# Autodesk Inventor assembly: b5
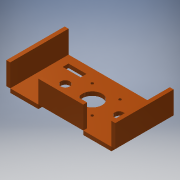
[picture p0: Inventor's stored thumbnail of the model, 180x180]
Saved by Autodesk Inventor 2017 (Build 210142000, 142)
## iProperties
Created: 2016-06-11
Part Number: b5
Document SubType Name: Assembly
Designer: daniel
Author: daniel
## Documents named in this file (4)
- C:\Users\daniel\Documents\GitHub\cardboard-stage-metric\stage\b5.iam
- C:\Users\daniel\Documents\GitHub\cardboard-stage-metric\stage\b3b.ipt
- C:\Users\daniel\Documents\GitHub\cardboard-stage-metric\stage\b3c.ipt
- C:\Users\daniel\Documents\GitHub\cardboard-stage-metric\stage\b5a.ipt
## Components (4 placed, 3 different names)
1. b5a:1 — Mate:1, Mate:2, Flush:1, Flush:2, Mate:3, Mate:4, Mate:5, Mate:6, Mate:7
2. b3b:1 — Mate:1, Flush:1, Mate:3
3. b3c:1 — Mate:5, Mate:6, Mate:7
4. b3b:2 — Mate:2, Flush:2, Mate:4
## Relationships (9: Mate 7, Flush 2)
- Mate:1: b5a:1 ↔ b3b:1
- Mate:2: b5a:1 ↔ b3b:2
- Flush:1: b5a:1 ↔ b3b:1
- Flush:2: b5a:1 ↔ b3b:2
- Mate:3: b5a:1 ↔ b3b:1
- Mate:4: b5a:1 ↔ b3b:2
- Mate:5: b5a:1 ↔ b3c:1
- Mate:6: b5a:1 ↔ b3c:1
- Mate:7: b5a:1 ↔ b3c:1
